# Autodesk Inventor assembly: Assembly_Rymapt_Ethoscope2
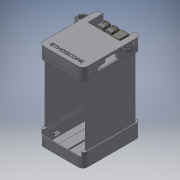
[picture p0: Inventor's stored thumbnail of the model, 180x180]
Saved by Autodesk Inventor 2017 (Build 210142000, 142)
## iProperties
Created: 2017-06-08
Part Number: Assembly_Rymapt_Ethoscope2
Document SubType Name: Assembly
Designer: Paolo
Author: Paolo
## Documents named in this file (12)
- E:\Rymapt_projects\Ethoscope\ethoscope_hardware\core_Rymapt\Assembly_Rymapt_Ethoscope2.iam
- E:\Rymapt_projects\Ethoscope\ethoscope_hardware\core_Rymapt\LightBox\core_lightBox_R2.ipt
- E:\Rymapt_projects\Ethoscope\ethoscope_hardware\core_Rymapt\PiCase\lowerPiCase_R2.ipt
- E:\Rymapt_projects\Ethoscope\ethoscope_hardware\core_Rymapt\PiCase\upperPiCase_R.ipt
- E:\Rymapt_projects\Ethoscope\ethoscope_hardware\core\RPi3\RasPi_Camera.ipt
- E:\Rymapt_projects\Ethoscope\ethoscope_hardware\extra\Screws\M2_phillip_8mm.ipt
- E:\Rymapt_projects\Ethoscope\ethoscope_hardware\core\RPi3\RPi3_ModelB.ipt
- E:\Rymapt_projects\Ethoscope\ethoscope_hardware\extra\Screws\M3_philips_6mm.ipt
- E:\Rymapt_projects\Ethoscope\ethoscope_hardware\extra\Screws\M3_hex_12mm.ipt
- E:\Rymapt_projects\Ethoscope\ethoscope_hardware\extra\Screws\M2_nut.ipt
- E:\Rymapt_projects\Ethoscope\ethoscope_hardware\core_Rymapt\LightBox\sideWall_R2.ipt
- E:\Rymapt_projects\Ethoscope\ethoscope_hardware\core_Rymapt\LightBox\core_lightStrip_R.ipt
## Components (18 placed, 11 different names)
1. core_lightBox_R2:1 — Flush:1, Flush:2, Mate:30, Mate:31, Mate:32, Mate:33, Mate:34, Mate:35, Mate:37, Mate:38, Mate:39, Mate:40
2. lowerPiCase_R2:1 — Flush:1, Flush:2, Mate:1, Mate:2, Mate:3, Mate:4, Mate:5, Mate:8, Mate:9, Mate:12, Mate:15, Mate:16, Mate:17, Mate:18, Mate:21, Mate:22, Mate:23, Mate:24, Mate:25, Mate:30, Mate:36
3. upperPiCase_R:1 — Mate:19, Mate:20, Mate:25
4. RasPi_Camera:1 — Mate:1, Mate:6, Mate:7, Mate:28, Mate:29
5. M2_phillip_8mm:1 — Mate:2, Mate:4, Mate:7, Mate:26
6. M2_phillip_8mm:2 — Mate:3, Mate:5, Mate:6, Mate:27
7. RPi3_ModelB:1 — Mate:8, Mate:10, Mate:11, Mate:13, Mate:14
8. M3_philips_6mm:1 — Mate:9, Mate:10, Mate:11
9. M3_philips_6mm:2 — Mate:12, Mate:13, Mate:14
10. M3_hex_12mm:1 — Mate:15, Mate:21
11. M3_hex_12mm:2 — Mate:16, Mate:19, Mate:22
12. M3_hex_12mm:3 — Mate:18, Mate:20, Mate:24
13. M3_hex_12mm:4 — Mate:17, Mate:23
14. M2_nut:1 — Mate:26, Mate:28
15. M2_nut:2 — Mate:27, Mate:29
16. sideWall_R2:1 — Mate:31, Mate:33, Mate:34, Mate:36
17. sideWall_R2:2 — Mate:32, Mate:35, Mate:37
18. core_lightStrip_R:1 — Mate:38, Mate:39, Mate:40
## Relationships (42: Mate 40, Flush 2)
- Flush:1: core_lightBox_R2:1 ↔ lowerPiCase_R2:1
- Flush:2: core_lightBox_R2:1 ↔ lowerPiCase_R2:1
- Mate:1: lowerPiCase_R2:1 ↔ RasPi_Camera:1
- Mate:2: lowerPiCase_R2:1 ↔ M2_phillip_8mm:1
- Mate:3: lowerPiCase_R2:1 ↔ M2_phillip_8mm:2
- Mate:4 (0.1 mm): lowerPiCase_R2:1 ↔ M2_phillip_8mm:1
- Mate:5 (0.1 mm): lowerPiCase_R2:1 ↔ M2_phillip_8mm:2
- Mate:6: RasPi_Camera:1 ↔ M2_phillip_8mm:2
- Mate:7: RasPi_Camera:1 ↔ M2_phillip_8mm:1
- Mate:8: lowerPiCase_R2:1 ↔ RPi3_ModelB:1
- Mate:9: lowerPiCase_R2:1 ↔ M3_philips_6mm:1
- Mate:10: RPi3_ModelB:1 ↔ M3_philips_6mm:1
- Mate:11 (0.1 mm): RPi3_ModelB:1 ↔ M3_philips_6mm:1
- Mate:12: lowerPiCase_R2:1 ↔ M3_philips_6mm:2
- Mate:13: RPi3_ModelB:1 ↔ M3_philips_6mm:2
- Mate:14 (0.1 mm): RPi3_ModelB:1 ↔ M3_philips_6mm:2
- Mate:15: lowerPiCase_R2:1 ↔ M3_hex_12mm:1
- Mate:16: lowerPiCase_R2:1 ↔ M3_hex_12mm:2
- Mate:17: lowerPiCase_R2:1 ↔ M3_hex_12mm:4
- Mate:18: lowerPiCase_R2:1 ↔ M3_hex_12mm:3
- Mate:19: upperPiCase_R:1 ↔ M3_hex_12mm:2
- Mate:20: upperPiCase_R:1 ↔ M3_hex_12mm:3
- Mate:21 (0.1 mm): lowerPiCase_R2:1 ↔ M3_hex_12mm:1
- Mate:22 (0.1 mm): lowerPiCase_R2:1 ↔ M3_hex_12mm:2
- Mate:23 (0.1 mm): lowerPiCase_R2:1 ↔ M3_hex_12mm:4
- Mate:24 (0.1 mm): lowerPiCase_R2:1 ↔ M3_hex_12mm:3
- Mate:25 (0.1 mm): lowerPiCase_R2:1 ↔ upperPiCase_R:1
- Mate:26: M2_phillip_8mm:1 ↔ M2_nut:1
- Mate:27: M2_phillip_8mm:2 ↔ M2_nut:2
- Mate:28 (0.1 mm): RasPi_Camera:1 ↔ M2_nut:1
- Mate:29 (0.1 mm): RasPi_Camera:1 ↔ M2_nut:2
- Mate:30 (130 mm): core_lightBox_R2:1 ↔ lowerPiCase_R2:1
- Mate:31 (0.1 mm): core_lightBox_R2:1 ↔ sideWall_R2:1
- Mate:32 (0.1 mm): core_lightBox_R2:1 ↔ sideWall_R2:2
- Mate:33 (0.1 mm): core_lightBox_R2:1 ↔ sideWall_R2:1
- Mate:34 (0.1 mm): core_lightBox_R2:1 ↔ sideWall_R2:1
- Mate:35 (0.1 mm): core_lightBox_R2:1 ↔ sideWall_R2:2
- Mate:36 (0.1 mm): lowerPiCase_R2:1 ↔ sideWall_R2:1
- Mate:37 (0.1 mm): core_lightBox_R2:1 ↔ sideWall_R2:2
- Mate:38 (0.1 mm): core_lightBox_R2:1 ↔ core_lightStrip_R:1
- Mate:39 (0.1 mm): core_lightBox_R2:1 ↔ core_lightStrip_R:1
- Mate:40 (0.1 mm): core_lightBox_R2:1 ↔ core_lightStrip_R:1
